# Autodesk Inventor assembly: !Drivebay Right
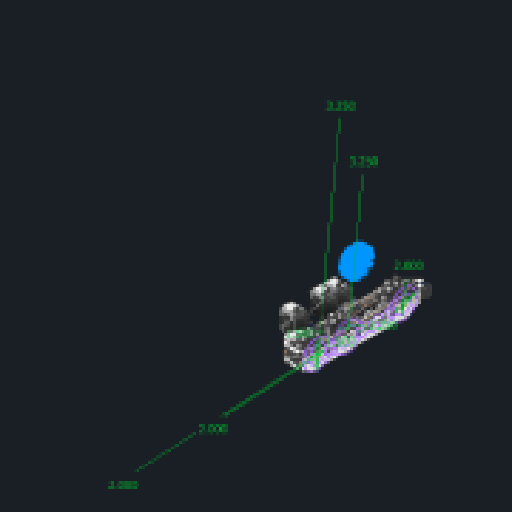
[picture p0: Inventor's stored thumbnail of the model, 512x512]
Saved by Autodesk Inventor 2025 (Build 290162000, 162)
## iProperties
Created: 2025-01-27
Part Number: !Drivebay Right
Document SubType Name: Assembly
Designer: Averey Ku
Author: Averey Ku
## Documents named in this file (10)
- D:\VEX\High Stakes\CAD\V5\Chassis\Drivebay Right\!Drivebay Right.iam
- D:\VEX\High Stakes\CAD\V5\Chassis\Drivebay Right\Outer.iam
- D:\VEX\High Stakes\CAD\V5\Chassis\Drivebay Right\Alu C 1x2x1x5.ipt
- D:\VEX\High Stakes\CAD\V5\Chassis\Drivebay Right\Inner.iam
- D:\VEX\High Stakes\CAD\V5\Chassis\Drivebay Right\Wheel.iam
- D:\VEX\High Stakes\CAD\V5\Chassis\Drivebay Right\Gear.iam
- D:\VEX\High Stakes\CAD\V5\Chassis\Drivebay Right\Ring Funnel.iam
- D:\VEX\High Stakes\CAD\V5\Chassis\Drivebay Right\MOGO Funnel.ipt
- D:\VEX\High Stakes\CAD\V5\Chassis\Drivebay Right\Skirt.ipt
- D:\VEX\High Stakes\CAD\ROBOPROS-CAD-Inventor\Structure\Nylon Standoff Rounded\Nylon Standoff 1.500.ipt
## Components (15 placed, 9 different names)
1. Outer:1 [sub-assembly] — Mate:1, Insert:1, Insert:3, Insert:4, Insert:5, Insert:6, Insert:7, Insert:8, Insert:9, Insert:10, Insert:11, Mate:4, Mate:5, Insert:12, Insert:13
2. Alu C 1x2x1x5:1 — Mate:1, Insert:1, Mate:2, Insert:2
3. Inner:1 [sub-assembly] — Mate:2, Insert:2, Mate:3
4. Wheel:1 [sub-assembly] — Insert:3
5. Wheel:2 [sub-assembly] — Insert:4
6. Wheel:3 [sub-assembly] — Insert:5
7. Gear:1 [sub-assembly] — Insert:6
8. Gear:2 [sub-assembly] — Insert:7
9. Gear:3 [sub-assembly] — Insert:8
10. Gear:4 [sub-assembly] — Insert:9
11. Ring Funnel:1 [sub-assembly] — Mate:3, Insert:10
12. MOGO Funnel:1 — Insert:11, Mate:4
13. MOGO Funnel:2 — Mate:5, Insert:12, Insert:14
14. Skirt:1 — Insert:13
15. Nylon Standoff 1.500:1 — Insert:14
## Relationships (19: Insert 14, Mate 5)
- Mate:1: Outer:1 ↔ Alu C 1x2x1x5:1
- Insert:1: Outer:1 ↔ Alu C 1x2x1x5:1
- Mate:2: Alu C 1x2x1x5:1 ↔ Inner:1
- Insert:2: Alu C 1x2x1x5:1 ↔ Inner:1
- Insert:3: Outer:1 ↔ Wheel:1
- Insert:4: Outer:1 ↔ Wheel:2
- Insert:5: Outer:1 ↔ Wheel:3
- Insert:6 (1.27 mm): Outer:1 ↔ Gear:1
- Insert:7 (1.27 mm): Outer:1 ↔ Gear:2
- Insert:8 (1.27 mm): Outer:1 ↔ Gear:3
- Insert:9 (1.27 mm): Outer:1 ↔ Gear:4
- Mate:3: Inner:1 ↔ Ring Funnel:1
- Insert:10: Outer:1 ↔ Ring Funnel:1
- Insert:11 (6.35 mm): Outer:1 ↔ MOGO Funnel:1
- Mate:4: Outer:1 ↔ MOGO Funnel:1
- Mate:5: Outer:1 ↔ MOGO Funnel:2
- Insert:12 (6.35 mm): Outer:1 ↔ MOGO Funnel:2
- Insert:13: Outer:1 ↔ Skirt:1
- Insert:14: MOGO Funnel:2 ↔ Nylon Standoff 1.500:1
